# Autodesk Inventor assembly: encoder_arr_1
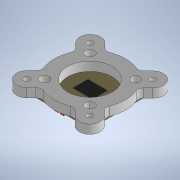
[picture p0: Inventor's stored thumbnail of the model, 180x180]
Saved by Autodesk Inventor 2020 (Build 240168000, 168)
## iProperties
Created: 2020-10-12
Part Number: encoder_arr_1
Document SubType Name: Assembly
Designer: Shuang Peng
Author: Shuang Peng
## Documents named in this file (3)
- D:\projects-3\biped_gen1\hardware\encoder_arr_1.iam
- D:\projects-3\biped_gen1\hardware\eletronic\encoder_as5047p v1\encoder_as5047p.iam
- D:\projects-3\biped_gen1\hardware\encoder_shelf_1.ipt
## Components (2 placed, 2 different names)
1. encoder_as5047p:1 [sub-assembly] — Flush:1
2. encoder_shelf_1:1 — Flush:1
## Relationships (1: Flush 1)
- Flush:1: encoder_as5047p:1 ↔ encoder_shelf_1:1
